# Autodesk Inventor assembly: onlyrobot
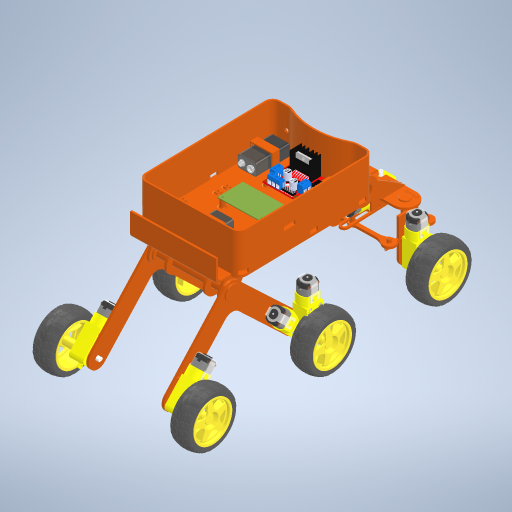
[picture p0: Inventor's stored thumbnail of the model, 512x512]
Saved by Autodesk Inventor 2023.2 (Build 272271000, 271)
## iProperties
Created: 2022-12-08
Part Number: onlyrobot
Document SubType Name: Assembly
Designer: omrfrkmll
Author: omrfrkmll
## Documents named in this file (27)
- C:\Users\omr_f\Desktop\mechanism design project\onlyrobot v2.iam
- C:\Users\omr_f\Desktop\mechanism design project\robotbase.ipt
- C:\Users\omr_f\Desktop\mechanism design project\sol arka bacak.ipt
- C:\Users\omr_f\Desktop\mechanism design project\6v dc torque motor.iam
- C:\Users\omr_f\Desktop\mechanism design project\Wheel D65x25.ipt
- C:\Users\omr_f\Desktop\mechanism design project\ön sol bacak.ipt
- C:\Users\omr_f\Desktop\mechanism design project\ön sol bacak_MIR.ipt
- C:\Users\omr_f\Desktop\mechanism design project\pin.ipt
- C:\Users\omr_f\Desktop\mechanism design project\pintutucu.ipt
- C:\Users\omr_f\Desktop\mechanism design project\pintutucu_MIR.ipt
- C:\Users\omr_f\Desktop\mechanism design project\dişli.ipt
- C:\Users\omr_f\Desktop\mechanism design project\rockerbogieçükü.ipt
- C:\Users\omr_f\Desktop\mechanism design project\6v dc torque motor_MIR.iam
- C:\Users\omr_f\Desktop\mechanism design project\Wheel D65x25_MIR.ipt
- C:\Users\omr_f\Desktop\mechanism design project\rockerbogieçükü_MIR.ipt
- C:\Users\omr_f\Desktop\mechanism design project\çıkçık.ipt
- C:\Users\omr_f\Desktop\mechanism design project\çıkçıkkarşılıkk.ipt
- C:\Users\omr_f\Desktop\mechanism design project\L298N Driver DC Motor.ipt
- C:\Users\omr_f\Desktop\mechanism design project\devre kartı.ipt
- C:\Users\omr_f\Desktop\mechanism design project\9 Volt Battery.ipt
- C:\Users\omr_f\Desktop\mechanism design project\direksiyon mili tutucu.ipt
- C:\Users\omr_f\Desktop\mechanism design project\şaftuzun.ipt
- C:\Users\omr_f\Desktop\mechanism design project\sol arka bacak_MIR.ipt
- C:\Users\omr_f\Desktop\mechanism design project\destek bağlantısı.ipt
- C:\Users\omr_f\Desktop\mechanism design project\steering system tutucu.ipt
- C:\Users\omr_f\Desktop\mechanism design project\steering rod.ipt
- C:\Users\omr_f\Desktop\mechanism design project\aksisde.ipt
## Components (47 placed, 26 different names)
1. robotbase:1 — Mate:87, Mate:88, Mate:89, Mate:90, Mate:91, Mate:92, Mate:94, Mate:95, Mate:96, Mate:97, Mate:99, Mate:100, Mate:101, Mate:102, Mate:103, Mate:113, Mate:114, Mate:115, Mate:120, Mate:121, Mate:122
2. 6v dc torque motor:1 [sub-assembly]
3. Wheel D65x25:1
4. ön sol bacak:1 — Mate:126, Mate:142, Mate:143, Mate:144
5. ön sol bacak_MIR:1 — Mate:133
6. 6v dc torque motor:2 [sub-assembly]
7. Wheel D65x25:2
8. pin:1 — Mate:136, Mate:138
9. pintutucu:1 — Mate:147, Mate:148, Mate:149, Mate:151
10. pintutucu_MIR:1 — Mate:146, Mate:150
11. pin:2 — Mate:137, Mate:139
12. 6v dc torque motor:3 [sub-assembly]
13. Wheel D65x25:3
14. dişli:1
15. rockerbogieçükü:1 — Mate:123
16. 6v dc torque motor:4 [sub-assembly]
17. Wheel D65x25:4
18. 6v dc torque motor_MIR:1 [sub-assembly]
19. Wheel D65x25_MIR:1
20. rockerbogieçükü_MIR:1 — Mate:118
21. 6v dc torque motor_MIR:2 [sub-assembly]
22. Wheel D65x25_MIR:2
23. çıkçık:1 — Mate:117, Mate:124
24. çıkçıkkarşılıkk:1 — Mate:107
25. L298N Driver DC Motor:1 — Mate:90, Mate:91
26. L298N Driver DC Motor:2 — Mate:87, Mate:88
27. L298N Driver DC Motor:3 — Mate:89, Mate:92
28. çıkçık:2
29. çıkçıkkarşılıkk:2 — Mate:116, Mate:119
30. devre kartı:1 — Mate:94, Mate:95, Mate:96
31. 9 Volt Battery:1 — Mate:97, Mate:101
32. direksiyon mili tutucu:1
33. 9 Volt Battery:2 — Mate:99, Mate:102
34. 9 Volt Battery:3 — Mate:100, Mate:103
35. şaftuzun:1 — Mate:107, Mate:116, Mate:117, Mate:124
36. sol arka bacak:1 — Mate:113, Mate:114, Mate:115, Mate:118, Mate:119
37. sol arka bacak_MIR:1 — Mate:120, Mate:121, Mate:122, Mate:123
38. çıkçık:3 — Mate:127
39. çıkçıkkarşılıkk:3 — Mate:126, Mate:127, Mate:135
40. destek bağlantısı:1 — Mate:135
41. destek bağlantısı:2 — Mate:133
42. 6v dc torque motor:5 [sub-assembly]
43. 6v dc torque motor:6 [sub-assembly] — Mate:140, Mate:141, Mate:145, Mate:152
44. steering system tutucu:1 — Mate:136, Mate:137, Mate:138, Mate:139, Mate:140, Mate:141, Mate:142, Mate:143, Mate:144, Mate:145
45. steering rod:1 — Mate:146, Mate:147, Mate:151
46. steering rod:2 — Mate:148, Mate:149, Mate:150, Mate:153
47. aksisde:1 — Mate:152, Mate:153
## Relationships (102: Mate 102)
- [Mate]: 6v dc torque motor:1 ↔ Wheel D65x25:1
- [Mate]: 6v dc torque motor:1 ↔ Wheel D65x25:1
- [Mate]: robotbase:1 ↔ ön sol bacak:1
- [Mate]: robotbase:1 ↔ ön sol bacak:1
- [Mate]: robotbase:1 ↔ ön sol bacak:1
- [Mate]: robotbase:1 ↔ ön sol bacak_MIR:1
- [Mate]: robotbase:1 ↔ ön sol bacak_MIR:1
- [Mate]: robotbase:1 ↔ ön sol bacak_MIR:1
- [Mate]: 6v dc torque motor:2 ↔ Wheel D65x25:2
- [Mate]: 6v dc torque motor:2 ↔ Wheel D65x25:2
- [Mate]: pin:1 ↔ pintutucu:1
- [Mate]: pin:1 ↔ pintutucu:1
- [Mate]: 6v dc torque motor:2 ↔ pintutucu:1
- [Mate]: pin:1 ↔ pintutucu:1
- [Mate]: 6v dc torque motor:2 ↔ pintutucu:1
- [Mate]: 6v dc torque motor:2 ↔ pintutucu:1
- [Mate]: pintutucu_MIR:1 ↔ pin:2
- [Mate]: pintutucu_MIR:1 ↔ pin:2
- [Mate]: pintutucu_MIR:1 ↔ pin:2
- [Mate]: 6v dc torque motor:3 ↔ Wheel D65x25:3
- [Mate]: 6v dc torque motor:3 ↔ Wheel D65x25:3
- [Mate]: pintutucu_MIR:1 ↔ 6v dc torque motor:3
- [Mate]: pintutucu_MIR:1 ↔ 6v dc torque motor:3
- [Mate]: pintutucu_MIR:1 ↔ 6v dc torque motor:3
- [Mate]: 6v dc torque motor:2 ↔ pintutucu:1
- [Mate]: 6v dc torque motor:2 ↔ pintutucu:1
- [Mate]: 6v dc torque motor:1 ↔ rockerbogieçükü:1
- [Mate]: 6v dc torque motor:1 ↔ rockerbogieçükü:1
- [Mate]: 6v dc torque motor:1 ↔ rockerbogieçükü:1
- [Mate]: 6v dc torque motor:4 ↔ Wheel D65x25:4
- [Mate]: 6v dc torque motor:4 ↔ Wheel D65x25:4
- [Mate]: rockerbogieçükü:1 ↔ 6v dc torque motor:4
- [Mate]: rockerbogieçükü:1 ↔ 6v dc torque motor:4
- [Mate]: rockerbogieçükü:1 ↔ 6v dc torque motor:4
- [Mate]: 6v dc torque motor_MIR:1 ↔ Wheel D65x25_MIR:1
- [Mate]: 6v dc torque motor_MIR:1 ↔ Wheel D65x25_MIR:1
- [Mate]: 6v dc torque motor_MIR:1 ↔ rockerbogieçükü_MIR:1
- [Mate]: 6v dc torque motor_MIR:1 ↔ rockerbogieçükü_MIR:1
- [Mate]: 6v dc torque motor_MIR:1 ↔ rockerbogieçükü_MIR:1
- [Mate]: rockerbogieçükü_MIR:1 ↔ 6v dc torque motor_MIR:2
- [Mate]: rockerbogieçükü_MIR:1 ↔ 6v dc torque motor_MIR:2
- [Mate]: rockerbogieçükü_MIR:1 ↔ 6v dc torque motor_MIR:2
- [Mate]: 6v dc torque motor_MIR:2 ↔ Wheel D65x25_MIR:2
- [Mate]: 6v dc torque motor_MIR:2 ↔ Wheel D65x25_MIR:2
- [Mate]: rockerbogieçükü:1 ↔ çıkçık:1
- [Mate]: rockerbogieçükü:1 ↔ çıkçık:1
- [Mate]: çıkçık:1 ↔ çıkçıkkarşılıkk:1
- [Mate]: rockerbogieçükü_MIR:1 ↔ çıkçık:2
- [Mate]: rockerbogieçükü_MIR:1 ↔ çıkçıkkarşılıkk:2
- [Mate]: rockerbogieçükü_MIR:1 ↔ çıkçık:2
- [Mate]: çıkçık:2 ↔ çıkçıkkarşılıkk:2
- Mate:87: robotbase:1 ↔ L298N Driver DC Motor:2
- Mate:88: robotbase:1 ↔ L298N Driver DC Motor:2
- Mate:89: robotbase:1 ↔ L298N Driver DC Motor:3
- Mate:90: robotbase:1 ↔ L298N Driver DC Motor:1
- Mate:91: robotbase:1 ↔ L298N Driver DC Motor:1
- Mate:92: robotbase:1 ↔ L298N Driver DC Motor:3
- Mate:94: robotbase:1 ↔ devre kartı:1
- Mate:95: robotbase:1 ↔ devre kartı:1
- Mate:96: robotbase:1 ↔ devre kartı:1
- Mate:97: robotbase:1 ↔ 9 Volt Battery:1
- Mate:99: robotbase:1 ↔ 9 Volt Battery:2
- Mate:100: robotbase:1 ↔ 9 Volt Battery:3
- Mate:101: robotbase:1 ↔ 9 Volt Battery:1
- Mate:102: robotbase:1 ↔ 9 Volt Battery:2
- Mate:103: robotbase:1 ↔ 9 Volt Battery:3
- Mate:107: çıkçıkkarşılıkk:1 ↔ şaftuzun:1
- Mate:113: robotbase:1 ↔ sol arka bacak:1
- Mate:114: robotbase:1 ↔ sol arka bacak:1
- Mate:115: robotbase:1 ↔ sol arka bacak:1
- Mate:116: çıkçıkkarşılıkk:2 ↔ şaftuzun:1
- Mate:117: çıkçık:1 ↔ şaftuzun:1
- Mate:118: rockerbogieçükü_MIR:1 ↔ sol arka bacak:1
- Mate:119: çıkçıkkarşılıkk:2 ↔ sol arka bacak:1
- Mate:120: robotbase:1 ↔ sol arka bacak_MIR:1
- Mate:121: robotbase:1 ↔ sol arka bacak_MIR:1
- Mate:122: robotbase:1 ↔ sol arka bacak_MIR:1
- Mate:123: rockerbogieçükü:1 ↔ sol arka bacak_MIR:1
- Mate:124 (2 mm): çıkçık:1 ↔ şaftuzun:1
- [Mate]: çıkçık:3 ↔ çıkçıkkarşılıkk:3
- Mate:126: ön sol bacak:1 ↔ çıkçıkkarşılıkk:3
- Mate:127: çıkçık:3 ↔ çıkçıkkarşılıkk:3
- Mate:133: ön sol bacak_MIR:1 ↔ destek bağlantısı:2
- Mate:135: çıkçıkkarşılıkk:3 ↔ destek bağlantısı:1
- Mate:136: pin:1 ↔ steering system tutucu:1
- Mate:137: pin:2 ↔ steering system tutucu:1
- Mate:138: pin:1 ↔ steering system tutucu:1
- Mate:139: pin:2 ↔ steering system tutucu:1
- Mate:140: 6v dc torque motor:6 ↔ steering system tutucu:1
- Mate:141 (1 mm): 6v dc torque motor:6 ↔ steering system tutucu:1
- Mate:142: ön sol bacak:1 ↔ steering system tutucu:1
- Mate:143: ön sol bacak:1 ↔ steering system tutucu:1
- Mate:144: ön sol bacak:1 ↔ steering system tutucu:1
- Mate:145: 6v dc torque motor:6 ↔ steering system tutucu:1
- Mate:146: pintutucu_MIR:1 ↔ steering rod:1
- Mate:147: pintutucu:1 ↔ steering rod:1
- Mate:148: pintutucu:1 ↔ steering rod:2
- Mate:149: pintutucu:1 ↔ steering rod:2
- Mate:150: pintutucu_MIR:1 ↔ steering rod:2
- Mate:151: pintutucu:1 ↔ steering rod:1
- Mate:152: 6v dc torque motor:6 ↔ aksisde:1
- Mate:153 (1 mm): steering rod:2 ↔ aksisde:1
## Named parameters: d156_d59_d45 = 0 mm, d157_d60_d46 = 0 mm, d100_d59_d45 = 0 mm, d101_d60_d46 = 0 mm, d59_d45 = 0 mm, d60_d46 = 0 mm, d59_d65 = 0 mm, d60_d68 = 0 mm, d61_d69 = 0 mm, d62_d70 = 0 mm, d63_d71 = 0 mm, d64_d72 = 0 mm, d77_d45 = 0 mm, d78_d46 = 0 mm, d72_d85 = 0 mm, d172_d196 = 0 mm
